# Autodesk Inventor assembly: maze_version1
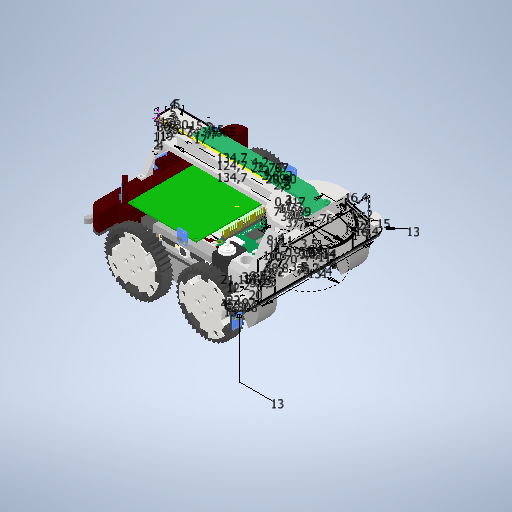
[picture p0: Inventor's stored thumbnail of the model, 512x512]
Saved by Autodesk Inventor 2025 (Build 290162000, 162)
## iProperties
Created: 2026-02-09
Part Number: maze_version1
Document SubType Name: Assembly
Designer: garin
Author: garin
## Documents named in this file (37)
- C:\Users\Leva\Documents\Git\Theseus_Maze\construction\version1\3D\maze_version1.iam
- C:\Users\Leva\Documents\Git\Theseus_Maze\construction\version1\3D\base.ipt
- C:\Users\Leva\Documents\Git\Theseus_Maze\construction\version1\3D\fast_battery.ipt
- C:\Users\Leva\Documents\Git\Theseus_Maze\construction\version1\3D\front_part_1.ipt
- C:\Users\Leva\Documents\Git\Theseus_Maze\construction\version1\3D\front_part_2.ipt
- C:\Users\Leva\Documents\Git\Theseus_Maze\construction\version1\3D\VL53L0X_TOF.ipt
- C:\Users\Leva\Documents\Git\Theseus_Maze\construction\version1\3D\fast_RGB.ipt
- C:\Users\Leva\Documents\Git\Theseus_Maze\construction\version1\3D\TCS34725 RGB sensor.ipt
- C:\Users\Leva\Documents\Git\Theseus_Maze\construction\version1\3D\end_cap.ipt
- C:\Users\Leva\Documents\Git\Theseus_Maze\construction\version1\3D\back_part.ipt
- C:\Users\Leva\Documents\Git\Theseus_Maze\construction\version1\3D\raspberry_pi_5.ipt
- C:\Users\Leva\Documents\Git\Theseus_Maze\construction\version1\3D\board.ipt
- C:\Users\Leva\Documents\Git\Theseus_Maze\construction\version1\3D\motor_25_110RPM.ipt
- C:\Users\Leva\Documents\Git\Theseus_Maze\construction\version1\3D\circle.ipt
- C:\Users\Leva\Documents\Git\Theseus_Maze\construction\version1\3D\колёса.ipt
- C:\Users\Leva\Documents\Git\Theseus_Maze\construction\version1\3D\fast_motors_left.ipt
- C:\Users\Leva\Documents\Git\Theseus_Maze\construction\version1\3D\fast_motors_right.ipt
- C:\Users\Leva\Documents\Git\Theseus_Maze\construction\version1\3D\fast_akkum.ipt
- C:\Users\Leva\Documents\Git\Theseus_Maze\construction\version1\3D\fast_akkum2.ipt
- C:\Users\Leva\Documents\Git\Theseus_Maze\construction\version1\3D\system_extrad.ipt
- C:\Users\Leva\Documents\Git\Theseus_Maze\construction\version1\3D\fast_camera.ipt
- C:\Users\Leva\Documents\Git\Theseus_Maze\construction\version1\3D\Arducam USB Camera module B0431.ipt
- C:\Users\Leva\Documents\Git\Theseus_Maze\construction\version1\3D\TOF VL53L0X.ipt
- C:\Users\Leva\Documents\Git\Theseus_Maze\construction\version1\3D\wheel.iam
- C:\Users\Leva\Documents\Git\Theseus_Maze\construction\version1\3D\COUPLE FLANGE.ipt
- C:\Users\Leva\Documents\Git\Theseus_Maze\construction\version1\3D\camera.ipt
- C:\Users\Leva\Documents\Git\Theseus_Maze\construction\version1\3D\fast_switch.ipt
- C:\Users\Leva\Documents\Git\Theseus_Maze\construction\version1\3D\Tumbler MT1.ipt
- C:\Users\Leva\Documents\Git\Theseus_Maze\construction\version1\3D\cube.ipt
- C:\Users\Leva\Documents\Git\Theseus_Maze\construction\version1\3D\akkum.iam
- C:\Users\Leva\Documents\Git\Theseus_Maze\construction\version1\3D\SSD1327.ipt
- C:\Users\Leva\Documents\Git\Theseus_Maze\construction\version1\stl\wire_fixs.ipt
- C:\Users\Leva\Documents\Git\Theseus_Maze\construction\version1\stl\cap_of _exstrad.ipt
- C:\Users\Leva\Documents\Git\Theseus_Maze\construction\version1\3D\new_back_part.ipt
- C:\Users\Leva\Documents\Git\Theseus_Maze\construction\version1\3D\new_extrad_system.ipt
- C:\Users\Leva\Documents\Git\Theseus_Maze\construction\version1\3D\handle.ipt
- C:\Users\Leva\Documents\Git\Theseus_Maze\construction\version1\3D\low_part_of_extrad_system.ipt
## Components (57 placed, 36 different names)
1. base:1 — Заподлицо:1, Заподлицо:2, Заподлицо:3, Заподлицо:4, С поворотом:5, Заподлицо:6, С поворотом:15, С поворотом:19, Заподлицо:10, С поворотом:21, Заподлицо:11, Заподлицо:12, Заподлицо:14, С поворотом:27, С поворотом:47, Заподлицо:15, Ползун:1, Заподлицо:17, Совмещение:1, Совмещение:2
2. fast_battery:1 — Заподлицо:1
3. front_part_1:1 — Заподлицо:2, С поворотом:6, Заподлицо:5, С поворотом:10, С поворотом:21
4. front_part_2:1 — Заподлицо:3, Заподлицо:4, С поворотом:6, С поворотом:7, С поворотом:8, С поворотом:11, С поворотом:14, С поворотом:28, С поворотом:29
5. fast_RGB:1 — С поворотом:5, С поворотом:9
6. VL53L0X_TOF:1 — С поворотом:7
7. VL53L0X_TOF:2 — С поворотом:8
8. TCS34725 RGB sensor:1 — С поворотом:9
9. end_cap:1 — Заподлицо:5
10. end_cap:2 — С поворотом:10
11. VL53L0X_TOF:3 — С поворотом:11
12. back_part:1 — Заподлицо:6, С поворотом:15, С поворотом:20, С поворотом:30, С поворотом:50, Жесткий:4
13. raspberry_pi_5:1 — Совмещение:3, Совмещение:4, Угол:1
14. board:1 — С поворотом:14
15. motor_25_110RPM:2 — С поворотом:36
16. motor_25_110RPM:3 — С поворотом:33
17. motor_25_110RPM:4 — С поворотом:34
18. motor_25_110RPM:5 — С поворотом:35
19. circle:1 — Заподлицо:13, Жесткий:3
20. колёса:1
21. fast_motors_left:1 — С поворотом:27
22. fast_motors_right:1 — С поворотом:19
23. VL53L0X_TOF:4 — С поворотом:20
24. fast_akkum:1 — Заподлицо:10
25. fast_akkum2:1 — Заподлицо:11, Заподлицо:16
26. system_extrad:1 — Заподлицо:12, Жесткий:4
27. fast_camera:1 — Заподлицо:14, Жесткий:1, С поворотом:31, С поворотом:42
28. fast_camera:2 — Жесткий:2, С поворотом:47, С поворотом:48
29. Arducam USB Camera module B0431:1 — Жесткий:1
30. Arducam USB Camera module B0431:2
31. TOF VL53L0X:1
32. TOF VL53L0X:2 — С поворотом:28
33. TOF VL53L0X:3 — С поворотом:29
34. TOF VL53L0X:4 — С поворотом:30
35. TOF VL53L0X:5 — С поворотом:31
36. TOF VL53L0X:6 — С поворотом:48
37. COUPLE FLANGE:1 — С поворотом:33, С поворотом:45
38. COUPLE FLANGE:2 — С поворотом:36, С поворотом:43
39. COUPLE FLANGE:3 — С поворотом:35, С поворотом:44
40. COUPLE FLANGE:4 — С поворотом:34, С поворотом:46
41. camera:1 — Жесткий:2
42. camera:2 — С поворотом:42
43. wheel:1 [sub-assembly] — С поворотом:43
44. wheel:2 [sub-assembly] — С поворотом:46
45. wheel:3 [sub-assembly] — С поворотом:45
46. wheel:4 [sub-assembly] — С поворотом:44
47. fast_switch:1 — Заподлицо:15, С поворотом:49
48. Tumbler MT1:1 — С поворотом:49
49. cube:1 — Жесткий:3
50. akkum:1 [sub-assembly] — Ползун:1
51. SSD1327:1 — С поворотом:50
52. wire_fixs:1 — Заподлицо:16
53. cap_of _exstrad:1
54. new_back_part:1 — Заподлицо:17, Совмещение:1, Совмещение:2, Совмещение:3, Совмещение:4, Угол:1, Совмещение:5
55. new_extrad_system:1 — Совмещение:5, Заподлицо:18, Совмещение:6, Совмещение:7, Совмещение:8
56. handle:1 — Заподлицо:18
57. low_part_of_extrad_system:1 — Совмещение:6, Совмещение:7, Совмещение:8
## Relationships (59: RevoluteJoint 30, Flush 15, Mate 8, WeldJoint 4, TranslationJoint 1, Angle 1)
- Заподлицо:1 [Flush]: base:1 ↔ fast_battery:1
- Заподлицо:2 [Flush]: base:1 ↔ front_part_1:1
- Заподлицо:3 [Flush]: base:1 ↔ front_part_2:1
- Заподлицо:4 [Flush] (9 mm): base:1 ↔ front_part_2:1
- С поворотом:5 [RevoluteJoint]: base:1 ↔ fast_RGB:1
- С поворотом:6 [RevoluteJoint]: front_part_1:1 ↔ front_part_2:1
- С поворотом:7 [RevoluteJoint]: front_part_2:1 ↔ VL53L0X_TOF:1
- С поворотом:8 [RevoluteJoint]: front_part_2:1 ↔ VL53L0X_TOF:2
- С поворотом:9 [RevoluteJoint]: fast_RGB:1 ↔ TCS34725 RGB sensor:1
- Заподлицо:5 [Flush]: front_part_1:1 ↔ end_cap:1
- С поворотом:10 [RevoluteJoint]: front_part_1:1 ↔ end_cap:2
- С поворотом:11 [RevoluteJoint]: front_part_2:1 ↔ VL53L0X_TOF:3
- Заподлицо:6 [Flush]: base:1 ↔ back_part:1
- С поворотом:14 [RevoluteJoint]: front_part_2:1 ↔ board:1
- С поворотом:15 [RevoluteJoint]: base:1 ↔ back_part:1
- С поворотом:19 [RevoluteJoint]: base:1 ↔ fast_motors_right:1
- С поворотом:20 [RevoluteJoint]: back_part:1 ↔ VL53L0X_TOF:4
- Заподлицо:10 [Flush]: base:1 ↔ fast_akkum:1
- С поворотом:21 [RevoluteJoint]: base:1 ↔ front_part_1:1
- Заподлицо:11 [Flush]: base:1 ↔ fast_akkum2:1
- Заподлицо:12 [Flush]: base:1 ↔ system_extrad:1
- Заподлицо:13 [Flush] (-1 mm): circle:1
- Заподлицо:14 [Flush]: base:1 ↔ fast_camera:1
- С поворотом:27 [RevoluteJoint]: base:1 ↔ fast_motors_left:1
- Жесткий:1 [WeldJoint]: fast_camera:1 ↔ Arducam USB Camera module B0431:1
- С поворотом:28 [RevoluteJoint]: front_part_2:1 ↔ TOF VL53L0X:2
- С поворотом:29 [RevoluteJoint]: front_part_2:1 ↔ TOF VL53L0X:3
- С поворотом:30 [RevoluteJoint]: back_part:1 ↔ TOF VL53L0X:4
- С поворотом:31 [RevoluteJoint]: fast_camera:1 ↔ TOF VL53L0X:5
- С поворотом:33 [RevoluteJoint]: motor_25_110RPM:3 ↔ COUPLE FLANGE:1
- С поворотом:34 [RevoluteJoint]: motor_25_110RPM:4 ↔ COUPLE FLANGE:4
- С поворотом:35 [RevoluteJoint]: motor_25_110RPM:5 ↔ COUPLE FLANGE:3
- С поворотом:36 [RevoluteJoint]: motor_25_110RPM:2 ↔ COUPLE FLANGE:2
- С поворотом:42 [RevoluteJoint]: fast_camera:1 ↔ camera:2
- Жесткий:2 [WeldJoint]: fast_camera:2 ↔ camera:1
- С поворотом:43 [RevoluteJoint]: COUPLE FLANGE:2 ↔ wheel:1
- С поворотом:44 [RevoluteJoint]: COUPLE FLANGE:3 ↔ wheel:4
- С поворотом:45 [RevoluteJoint]: COUPLE FLANGE:1 ↔ wheel:3
- С поворотом:46 [RevoluteJoint]: COUPLE FLANGE:4 ↔ wheel:2
- С поворотом:47 [RevoluteJoint]: base:1 ↔ fast_camera:2
- С поворотом:48 [RevoluteJoint]: fast_camera:2 ↔ TOF VL53L0X:6
- Заподлицо:15 [Flush]: base:1 ↔ fast_switch:1
- С поворотом:49 [RevoluteJoint]: fast_switch:1 ↔ Tumbler MT1:1
- Жесткий:3 [WeldJoint]: circle:1 ↔ cube:1
- Ползун:1 [TranslationJoint] (12 mm): base:1 ↔ akkum:1
- С поворотом:50 [RevoluteJoint]: back_part:1 ↔ SSD1327:1
- Заподлицо:16 [Flush]: fast_akkum2:1 ↔ wire_fixs:1
- Жесткий:4 [WeldJoint]: back_part:1 ↔ system_extrad:1
- Заподлицо:17 [Flush]: base:1 ↔ new_back_part:1
- Совмещение:1 [Mate]: base:1 ↔ new_back_part:1
- Совмещение:2 [Mate]: base:1 ↔ new_back_part:1
- Совмещение:3 [Mate]: raspberry_pi_5:1 ↔ new_back_part:1
- Совмещение:4 [Mate]: raspberry_pi_5:1 ↔ new_back_part:1
- Угол:1 [Angle] (180 deg): raspberry_pi_5:1 ↔ new_back_part:1
- Совмещение:5 [Mate]: new_back_part:1 ↔ new_extrad_system:1
- Заподлицо:18 [Flush]: new_extrad_system:1 ↔ handle:1
- Совмещение:6 [Mate]: new_extrad_system:1 ↔ low_part_of_extrad_system:1
- Совмещение:7 [Mate]: new_extrad_system:1 ↔ low_part_of_extrad_system:1
- Совмещение:8 [Mate]: new_extrad_system:1 ↔ low_part_of_extrad_system:1
